# Autodesk Inventor assembly: ring-holder
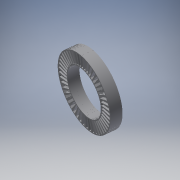
[picture p0: Inventor's stored thumbnail of the model, 180x180]
Saved by Autodesk Inventor 2018 (Build 220112000, 112)
## iProperties
Created: 2024-05-02
Part Number: ring-holder
Document SubType Name: Assembly
Designer: neo
Author: neo
## Documents named in this file (2)
- D:\projects\kreion\design1\3d\ring-holder.iam
- D:\projects\kreion\design1\3d\ring-holder-one-sixth.iam
## Components (6 placed, 1 different names)
1. ring-holder-one-sixth:1 [sub-assembly] — Flush:1, Flush:2, Mate:3, Mate:4, Tangent:3, Tangent:4, Tangent:5, Flush:5
2. ring-holder-one-sixth:2 [sub-assembly] — Flush:1, Mate:3, Tangent:5, Mate:5, Tangent:6
3. ring-holder-one-sixth:3 [sub-assembly] — Flush:2, Mate:4, Tangent:3, Tangent:4
4. ring-holder-one-sixth:4 [sub-assembly] — Flush:4, Mate:1, Tangent:1, Mate:5, Tangent:6
5. ring-holder-one-sixth:5 [sub-assembly] — Flush:3, Flush:4, Mate:1, Tangent:1, Mate:2, Tangent:2
6. ring-holder-one-sixth:6 [sub-assembly] — Flush:3, Mate:2, Tangent:2, Flush:5
## Relationships (16: Tangent 6, Flush 5, Mate 5)
- Flush:1: ring-holder-one-sixth:1 ↔ ring-holder-one-sixth:2
- Flush:2: ring-holder-one-sixth:1 ↔ ring-holder-one-sixth:3
- Flush:3: ring-holder-one-sixth:5 ↔ ring-holder-one-sixth:6
- Flush:4: ring-holder-one-sixth:4 ↔ ring-holder-one-sixth:5
- Mate:1: ring-holder-one-sixth:4 ↔ ring-holder-one-sixth:5
- Tangent:1: ring-holder-one-sixth:4 ↔ ring-holder-one-sixth:5
- Mate:2: ring-holder-one-sixth:5 ↔ ring-holder-one-sixth:6
- Tangent:2: ring-holder-one-sixth:5 ↔ ring-holder-one-sixth:6
- Mate:3: ring-holder-one-sixth:1 ↔ ring-holder-one-sixth:2
- Mate:4: ring-holder-one-sixth:1 ↔ ring-holder-one-sixth:3
- Tangent:3: ring-holder-one-sixth:1 ↔ ring-holder-one-sixth:3
- Tangent:4: ring-holder-one-sixth:1 ↔ ring-holder-one-sixth:3
- Tangent:5: ring-holder-one-sixth:1 ↔ ring-holder-one-sixth:2
- Flush:5: ring-holder-one-sixth:1 ↔ ring-holder-one-sixth:6
- Mate:5: ring-holder-one-sixth:2 ↔ ring-holder-one-sixth:4
- Tangent:6: ring-holder-one-sixth:2 ↔ ring-holder-one-sixth:4
